# Autodesk Inventor assembly: Assembly1
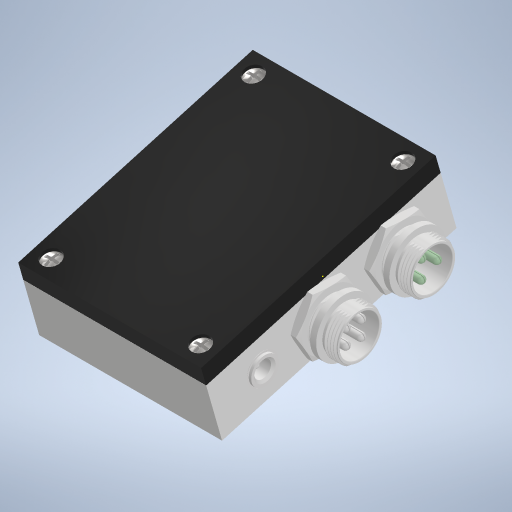
[picture p0: Inventor's stored thumbnail of the model, 512x512]
Saved by Autodesk Inventor 2023 (Build 270158000, 158)
## iProperties
Created: 2024-10-13
Part Number: Assembly1
Document SubType Name: Assembly
Designer: Juan
Author: Juan
## Documents named in this file (7)
- C:\Users\Juan\Documents\Inventor\Assembly1.iam
- C:\Users\Juan\Documents\Inventor\IOT2.ipt
- C:\Users\Juan\Documents\Inventor\Content Center Files\R2023\en-US\AS 1427(05)\AS 1427 - M5 x 6(5) II.ipt
- C:\Users\Juan\Downloads\dc-power-jack-2-1mm-socket-female-panel-mount-1.snapshot.2\DJ Jack 2,1mm panel mount.ipt
- C:\Users\Juan\Downloads\gx-16-connector-4-pins-1.snapshot.3\GX-16 Connector 4 Pins.iam
- C:\Users\Juan\Downloads\gx-16-connector-3-pins-1.snapshot.3\GX-16 Connector 3 Pins.iam
- D:\Semester 5\IoT dan Jaringan Sensor\aquasmart\aquasmart\aquasmart.iam
## Components (9 placed, 6 different names)
1. IOT2:1 — Mate:1, Mate:2, Mate:3, Mate:4, Mate:5, Mate:6, Mate:7, Mate:8, Insert:2, Insert:3, Flush:1, Mate:9
2. AS 1427 H - Metric M5 x 6:1 — Mate:1, Mate:2
3. AS 1427 H - Metric M5 x 6:2 — Mate:3, Mate:4
4. AS 1427 H - Metric M5 x 6:3 — Mate:5, Mate:6
5. AS 1427 H - Metric M5 x 6:4 — Mate:7, Mate:8
6. GX-16 Connector 4 Pins:1 [sub-assembly] — Insert:2
7. GX-16 Connector 3 Pins:1 [sub-assembly] — Insert:3
8. aquasmart:1 [sub-assembly] — Flush:1
9. DJ Jack 2,1mm panel mount:1 — Mate:9
## Relationships (12: Mate 9, Insert 2, Flush 1)
- Mate:1: IOT2:1 ↔ AS 1427 H - Metric M5 x 6:1
- Mate:2: IOT2:1 ↔ AS 1427 H - Metric M5 x 6:1
- Mate:3: IOT2:1 ↔ AS 1427 H - Metric M5 x 6:2
- Mate:4: IOT2:1 ↔ AS 1427 H - Metric M5 x 6:2
- Mate:5: IOT2:1 ↔ AS 1427 H - Metric M5 x 6:3
- Mate:6: IOT2:1 ↔ AS 1427 H - Metric M5 x 6:3
- Mate:7: IOT2:1 ↔ AS 1427 H - Metric M5 x 6:4
- Mate:8: IOT2:1 ↔ AS 1427 H - Metric M5 x 6:4
- Insert:2: IOT2:1 ↔ GX-16 Connector 4 Pins:1
- Insert:3: IOT2:1 ↔ GX-16 Connector 3 Pins:1
- Flush:1 (-12.7 mm): IOT2:1 ↔ aquasmart:1
- Mate:9: IOT2:1 ↔ DJ Jack 2,1mm panel mount:1
